(part 1 of 2)
# Autodesk Inventor assembly: Pauk
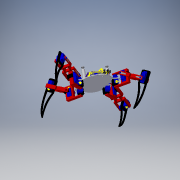
[picture p0: Inventor's stored thumbnail of the model, 180x180]
Saved by Autodesk Inventor 2019 (Build 230136000, 136)
## iProperties
Created: 2018-11-25
Part Number: Pauk
Document SubType Name: Assembly
Designer: nikol
_MechatronicsProject: <Project Version="1.0"><Path>C:\Users\nikol\Desktop\el.emx</Path><Guid>{C559D3A1-3329-4734-BE8F-63649D4C72C8}</Guid><IPJFileName>C:\Users\Public\Documents\Autodesk\Inventor 2019\Default.ipj</IPJFileName><IPJWorkFolder></IPJWorkFolder><AssemblyFileName>C:\Users\nikol\Desktop\ArduinoSpider\Modeli\Pauk.iam</AssemblyFileName><AssemblyFileGUID>{1F7FCD52-C9F9-4255-BD89-D36AF9ACCA5F}</AssemblyFileGUID></Project>
_MTAssemblyInfoProperty: <MechatronicsAssembly Version="1.0" ID="{1F7FCD52-C9F9-4255-BD89-D36AF9ACCA5F}"><MechatronicsComponents><MechatronicsComponent FileName="C:\Users\nikol\Desktop\ArduinoSpider\Modeli\SERVOMOTORARDUINO.ipt"><ReferenceKey Document="C:\Users\nikol\Desktop\ArduinoSpider\Modeli\Pauk.iam" Value="2|1|1|0|4|0|0|0|35|0|0|0|" Context="2|0|0|0|1|0|0|0|" ID="{1F7FCD52-C9F9-4255-BD89-D36AF9ACCA5F}"/><Properties><ComponentTag>(SERVOMOTORARDUINO:14)</ComponentTag><TerminalStripTag></TerminalStripTag><TerminalNumberTag></TerminalNumberTag><Installation></Installation><Location></Location><Category></Category><Manufacture></Manufacture><Catalog></Catalog><AssemblyCode></AssemblyCode><Line1></Line1><Line2></Line2><Line3></Line3><ElectricalType></ElectricalType></Properties><OccurrencePath><Occurrence Name="SERVOMOTORARDUINO:14" FileName="C:\Users\nikol\Desktop\ArduinoSpider\Modeli\SERVOMOTORARDUINO.ipt"/></OccurrencePath></MechatronicsComponent><MechatronicsComponent FileName="C:\Users\nikol\Desktop\ArduinoSpider\Modeli\SERVOMOTORARDUINO.ipt"><ReferenceKey Document="C:\Users\nikol\Desktop\ArduinoSpider\Modeli\Pauk.iam" Value="2|1|1|0|4|0|0|0|34|0|0|0|" Context="2|0|0|0|1|0|0|0|" ID="{1F7FCD52-C9F9-4255-BD89-D36AF9ACCA5F}"/><Properties><ComponentTag>(SERVOMOTORARDUINO:13)</ComponentTag><TerminalStripTag></TerminalStripTag><TerminalNumberTag></TerminalNumberTag><Installation></Installation><Location></Location><Category></Category><Manufacture></Manufacture><Catalog></Catalog><AssemblyCode></AssemblyCode><Line1></Line1><Line2></Line2><Line3></Line3><ElectricalType></ElectricalType></Properties><OccurrencePath><Occurrence Name="SERVOMOTORARDUINO:13" FileName="C:\Users\nikol\Desktop\ArduinoSpider\Modeli\SERVOMOTORARDUINO.ipt"/></OccurrencePath></MechatronicsComponent><MechatronicsComponent FileName="C:\Users\nikol\Desktop\ArduinoSpider\Modeli\SERVOMOTORARDUINO.ipt"><ReferenceKey Document="C:\Users\nikol\Desktop\ArduinoSpider\Modeli\Pauk.iam" Value="2|1|1|0|4|0|0|0|33|0|0|0|" Context="2|0|0|0|1|0|0|0|" ID="{1F7FCD52-C9F9-4255-BD89-D36AF9ACCA5F}"/><Properties><ComponentTag>(SERVOMOTORARDUINO:12)</ComponentTag><TerminalStripTag></TerminalStripTag><TerminalNumberTag></TerminalNumberTag><Installation></Installation><Location></Location><Category></Category><Manufacture></Manufacture><Catalog></Catalog><AssemblyCode></AssemblyCode><Line1></Line1><Line2></Line2><Line3></Line3><ElectricalType></ElectricalType></Properties><OccurrencePath><Occurrence Name="SERVOMOTORARDUINO:12" FileName="C:\Users\nikol\Desktop\ArduinoSpider\Modeli\SERVOMOTORARDUINO.ipt"/></OccurrencePath></MechatronicsComponent><MechatronicsComponent FileName="C:\Users\nikol\Desktop\ArduinoSpider\Modeli\SERVOMOTORARDUINO.ipt"><ReferenceKey Document="C:\Users\nikol\Desktop\ArduinoSpider\Modeli\Pauk.iam" Value="2|1|1|0|4|0|0|0|32|0|0|0|" Context="2|0|0|0|1|0|0|0|" ID="{1F7FCD52-C9F9-4255-BD89-D36AF9ACCA5F}"/><Properties><ComponentTag>(SERVOMOTORARDUINO:11)</ComponentTag><TerminalStripTag></TerminalStripTag><TerminalNumberTag></TerminalNumberTag><Installation></Installation><Location></Location><Category></Category><Manufacture></Manufacture><Catalog></Catalog><AssemblyCode></AssemblyCode><Line1></Line1><Line2></Line2><Line3></Line3><ElectricalType></ElectricalType></Properties><OccurrencePath><Occurrence Name="SERVOMOTORARDUINO:11" FileName="C:\Users\nikol\Desktop\ArduinoSpider\Modeli\SERVOMOTORARDUINO.ipt"/></OccurrencePath></MechatronicsComponent><MechatronicsComponent FileName="C:\Users\nikol\Desktop\ArduinoSpider\Modeli\SERVOMOTORARDUINO.ipt"><ReferenceKey Document="C:\Users\nikol\Desktop\ArduinoSpider\Modeli\Pauk.iam" Value="2|1|1|0|4|0|0|0|31|0|0|0|" Context="2|0|0|0|1|0|0|0|" ID="{1F7FCD52-C9F9-4255-BD89-D36AF9ACCA5F}"/><Properties><ComponentTag>(SERVOMOTORARDUINO:10)</ComponentTag><TerminalStripTag></TerminalStripTag><TerminalNumberTag></TerminalNumberTag><Installation></Installation><Location></Location><Category></Category><Manufacture></Manufacture><Catalog></Catalog><AssemblyCode></AssemblyCode><Line1></Line1><Line2></Line2><Line3></Line3><ElectricalType></ElectricalType></Properties><OccurrencePath><Occurrence Name="SERVOMOTORARDUINO:10" FileName="C:\Users\nikol\Desktop\ArduinoSpider\Modeli\SERVOMOTORARDUINO.ipt"/></OccurrencePath></MechatronicsComponent><MechatronicsComponent FileName="C:\Users\nikol\Desktop\ArduinoSpider\Modeli\SERVOMOTORARDUINO.ipt"><ReferenceKey Document="C:\Users\nikol\Desktop\ArduinoSpider\Modeli\Pauk.iam" Value="2|1|1|0|4|0|0|0|22|0|0|0|" Context="2|0|0|0|1|0|0|0|" ID="{1F7FCD52-C9F9-4255-BD89-D36AF9ACCA5F}"/><Properties><ComponentTag>(SERVOMOTORARDUINO:9)</ComponentTag><TerminalStripTag></TerminalStripTag><TerminalNumberTag></TerminalNumberTag><Installation></Installation><Location></Location><Category></Category><Manufacture></Manufacture><Catalog></Catalog><AssemblyCode></AssemblyCode><Line1></Line1><Line2></Line2><Line3></Line3><ElectricalType></ElectricalType></Properties><OccurrencePath><Occurrence Name="SERVOMOTORARDUINO:9" FileName="C:\Users\nikol\Desktop\ArduinoSpider\Modeli\SERVOMOTORARDUINO.ipt"/></OccurrencePath></MechatronicsComponent><MechatronicsComponent FileName="C:\Users\nikol\Desktop\ArduinoSpider\Modeli\SERVOMOTORARDUINO.ipt"><ReferenceKey Document="C:\Users\nikol\Desktop\ArduinoSpider\Modeli\Pauk.iam" Value="2|1|1|0|4|0|0|0|21|0|0|0|" Context="2|0|0|0|1|0|0|0|" ID="{1F7FCD52-C9F9-4255-BD89-D36AF9ACCA5F}"/><Properties><ComponentTag>(SERVOMOTORARDUINO:8)</ComponentTag><TerminalStripTag></TerminalStripTag><TerminalNumberTag></TerminalNumberTag><Installation></Installation><Location></Location><Category></Category><Manufacture></Manufacture><Catalog></Catalog><AssemblyCode></AssemblyCode><Line1></Line1><Line2></Line2><Line3></Line3><ElectricalType></ElectricalType></Properties><OccurrencePath><Occurrence Name="SERVOMOTORARDUINO:8" FileName="C:\Users\nikol\Desktop\ArduinoSpider\Modeli\SERVOMOTORARDUINO.ipt"/></OccurrencePath></MechatronicsComponent><MechatronicsComponent FileName="C:\Users\nikol\Desktop\ArduinoSpider\Modeli\SERVOMOTORARDUINO.ipt"><ReferenceKey Document="C:\Users\nikol\Desktop\ArduinoSpider\Modeli\Pauk.iam" Value="2|1|1|0|4|0|0|0|20|0|0|0|" Context="2|0|0|0|1|0|0|0|" ID="{1F7FCD52-C9F9-4255-BD89-D36AF9ACCA5F}"/><Properties><ComponentTag>(SERVOMOTORARDUINO:7)</ComponentTag><TerminalStripTag></TerminalStripTag><TerminalNumberTag></TerminalNumberTag><Installation></Installation><Location></Location><Category></Category><Manufacture></Manufacture><Catalog></Catalog><AssemblyCode></AssemblyCode><Line1></Line1><Line2></Line2><Line3></Line3><ElectricalType></ElectricalType></Properties><OccurrencePath><Occurrence Name="SERVOMOTORARDUINO:7" FileName="C:\Users\nikol\Desktop\ArduinoSpider\Modeli\SERVOMOTORARDUINO.ipt"/></OccurrencePath></MechatronicsComponent><MechatronicsComponent FileName="C:\Users\nikol\Desktop\ArduinoSpider\Modeli\SERVOMOTORARDUINO.ipt"><ReferenceKey Document="C:\Users\nikol\Desktop\ArduinoSpider\Modeli\Pauk.iam" Value="2|1|1|0|4|0|0|0|2|0|0|0|" Context="2|0|0|0|1|0|0|0|" ID="{1F7FCD52-C9F9-4255-BD89-D36AF9ACCA5F}"/><Properties><ComponentTag>(SERVOMOTORARDUINO:1)</ComponentTag><TerminalStripTag></TerminalStripTag><TerminalNumberTag></TerminalNumberTag><Installation></Installation><Location></Location><Category></Category><Manufacture></Manufacture><Catalog></Catalog><AssemblyCode></AssemblyCode><Line1></Line1><Line2></Line2><Line3></Line3><ElectricalType></ElectricalType></Properties><OccurrencePath><Occurrence Name="SERVOMOTORARDUINO:1" FileName="C:\Users\nikol\Desktop\ArduinoSpider\Modeli\SERVOMOTORARDUINO.ipt"/></OccurrencePath></MechatronicsComponent><MechatronicsComponent FileName="C:\Users\nikol\Desktop\ArduinoSpider\Modeli\SERVOMOTORARDUINO.ipt"><ReferenceKey Document="C:\Users\nikol\Desktop\ArduinoSpider\Modeli\Pauk.iam" Value="2|1|1|0|4|0|0|0|3|0|0|0|" Context="2|0|0|0|1|0|0|0|" ID="{1F7FCD52-C9F9-4255-BD89-D36AF9ACCA5F}"/><Properties><ComponentTag>(SERVOMOTORARDUINO:2)</ComponentTag><TerminalStripTag></TerminalStripTag><TerminalNumberTag></TerminalNumberTag><Installation></Installation><Location></Location><Category></Category><Manufacture></Manufacture><Catalog></Catalog><AssemblyCode></AssemblyCode><Line1></Line1><Line2></Line2><Line3></Line3><ElectricalType></ElectricalType></Properties><OccurrencePath><Occurrence Name="SERVOMOTORARDUINO:2" FileName="C:\Users\nikol\Desktop\ArduinoSpider\Modeli\SERVOMOTORARDUINO.ipt"/></OccurrencePath></MechatronicsComponent><MechatronicsComponent FileName="C:\Users\nikol\Desktop\ArduinoSpider\Modeli\SERVOMOTORARDUINO.ipt"><ReferenceKey Document="C:\Users\nikol\Desktop\ArduinoSpider\Modeli\Pauk.iam" Value="2|1|1|0|4|0|0|0|4|0|0|0|" Context="2|0|0|0|1|0|0|0|" ID="{1F7FCD52-C9F9-4255-BD89-D36AF9ACCA5F}"/><Properties><ComponentTag>(SERVOMOTORARDUINO:3)</ComponentTag><TerminalStripTag></TerminalStripTag><TerminalNumberTag></TerminalNumberTag><Installation></Installation><Location></Location><Category></Category><Manufacture></Manufacture><Catalog></Catalog><AssemblyCode></AssemblyCode><Line1></Line1><Line2></Line2><Line3></Line3><ElectricalType></ElectricalType></Properties><OccurrencePath><Occurrence Name="SERVOMOTORARDUINO:3" FileName="C:\Users\nikol\Desktop\ArduinoSpider\Modeli\SERVOMOTORARDUINO.ipt"/></OccurrencePath></MechatronicsComponent><MechatronicsComponent FileName="C:\Users\nikol\Desktop\ArduinoSpider\Modeli\SERVOMOTORARDUINO.ipt"><ReferenceKey Document="C:\Users\nikol\Desktop\ArduinoSpider\Modeli\Pauk.iam" Value="2|1|1|0|4|0|0|0|5|0|0|0|" Context="2|0|0|0|1|0|0|0|" ID="{1F7FCD52-C9F9-4255-BD89-D36AF9ACCA5F}"/><Properties><ComponentTag>(SERVOMOTORARDUINO:4)</ComponentTag><TerminalStripTag></TerminalStripTag><TerminalNumberTag></TerminalNumberTag><Installation></Installation><Location></Location><Category></Category><Manufacture></Manufacture><Catalog></Catalog><AssemblyCode></AssemblyCode><Line1></Line1><Line2></Line2><Line3></Line3><ElectricalType></ElectricalType></Properties><OccurrencePath><Occurrence Name="SERVOMOTORARDUINO:4" FileName="C:\Users\nikol\Desktop\ArduinoSpider\Modeli\SERVOMOTORARDUINO.ipt"/></OccurrencePath></MechatronicsComponent><MechatronicsComponent FileName="C:\Users\nikol\Desktop\ArduinoSpider\Modeli\Pertinaks.ipt"><ReferenceKey Document="C:\Users\nikol\Desktop\ArduinoSpider\Modeli\Pauk.iam" Value="2|1|1|0|4|0|0|0|70|0|0|0|" Context="2|0|0|0|1|0|0|0|" ID="{1F7FCD52-C9F9-4255-BD89-D36AF9ACCA5F}"/><Properties><ComponentTag>(Pertinaks:1)</ComponentTag><TerminalStripTag></TerminalStripTag><TerminalNumberTag></TerminalNumberTag><Installation></Installation><Location></Location><Category></Category><Manufacture></Manufacture><Catalog></Catalog><AssemblyCode></AssemblyCode><Line1></Line1><Line2></Line2><Line3></Line3><ElectricalType></ElectricalType></Properties><OccurrencePath><Occurrence Name="Pertinaks:1" FileName="C:\Users\nikol\Desktop\ArduinoSpider\Modeli\Pertinaks.ipt"/></OccurrencePath></MechatronicsComponent><MechatronicsComponent FileName="C:\Users\nikol\Desktop\ArduinoSpider\Modeli\Arduino1.ipt"><ReferenceKey Document="C:\Users\nikol\Desktop\ArduinoSpider\Modeli\Pauk.iam" Value="2|1|1|0|4|0|0|0|71|0|0|0|" Context="2|0|0|0|1|0|0|0|" ID="{1F7FCD52-C9F9-4255-BD89-D36AF9ACCA5F}"/><Properties><ComponentTag>(Arduino1:1)</ComponentTag><TerminalStripTag></TerminalStripTag><TerminalNumberTag></TerminalNumberTag><Installation></Installation><Location></Location><Category></Category><Manufacture></Manufacture><Catalog></Catalog><AssemblyCode></AssemblyCode><Line1></Line1><Line2></Line2><Line3></Line3><ElectricalType></ElectricalType></Properties><OccurrencePath><Occurrence Name="Arduino1:1" FileName="C:\Users\nikol\Desktop\ArduinoSpider\Modeli\Arduino1.ipt"/></OccurrencePath></MechatronicsComponent><MechatronicsComponent FileName="C:\Users\nikol\Desktop\ArduinoSpider\Modeli\konektorservomotora.ipt"><ReferenceKey Document="C:\Users\nikol\Desktop\ArduinoSpider\Modeli\Pauk.iam" Value="2|1|1|0|4|0|0|0|75|0|0|0|" Context="2|0|0|0|1|0|0|0|" ID="{1F7FCD52-C9F9-4255-BD89-D36AF9ACCA5F}"/><Properties><ComponentTag>(konektorservomotora:1)</ComponentTag><TerminalStripTag></TerminalStripTag><TerminalNumberTag></TerminalNumberTag><Installation></Installation><Location></Location><Category></Category><Manufacture></Manufacture><Catalog></Catalog><AssemblyCode></AssemblyCode><Line1></Line1><Line2></Line2><Line3></Line3><ElectricalType></ElectricalType></Properties><OccurrencePath><Occurrence Name="konektorservomotora:1" FileName="C:\Users\nikol\Desktop\ArduinoSpider\Modeli\konektorservomotora.ipt"/></OccurrencePath></MechatronicsComponent><MechatronicsComponent FileName="C:\Users\nikol\Desktop\ArduinoSpider\Modeli\konektorservomotora.ipt"><ReferenceKey Document="C:\Users\nikol\Desktop\ArduinoSpider\Modeli\Pauk.iam" Value="2|1|1|0|4|0|0|0|76|0|0|0|" Context="2|0|0|0|1|0|0|0|" ID="{1F7FCD52-C9F9-4255-BD89-D36AF9ACCA5F}"/><Properties><ComponentTag>(konektorservomotora:2)</ComponentTag><TerminalStripTag></TerminalStripTag><TerminalNumberTag></TerminalNumberTag><Installation></Installation><Location></Location><Category></Category><Manufacture></Manufacture><Catalog></Catalog><AssemblyCode></AssemblyCode><Line1></Line1><Line2></Line2><Line3></Line3><ElectricalType></ElectricalType></Properties><OccurrencePath><Occurrence Name="konektorservomotora:2" FileName="C:\Users\nikol\Desktop\ArduinoSpider\Modeli\konektorservomotora.ipt"/></OccurrencePath></MechatronicsComponent><MechatronicsComponent FileName="C:\Users\nikol\Desktop\ArduinoSpider\Modeli\konektorservomotora.ipt"><ReferenceKey Document="C:\Users\nikol\Desktop\ArduinoSpider\Modeli\Pauk.iam" Value="2|1|1|0|4|0|0|0|78|0|0|0|" Context="2|0|0|0|1|0|0|0|" ID="{1F7FCD52-C9F9-4255-BD89-D36AF9ACCA5F}"/><Properties><ComponentTag>(konektorservomotora:3)</ComponentTag><TerminalStripTag></TerminalStripTag><TerminalNumberTag></TerminalNumberTag><Installation></Installation><Location></Location><Category></Category><Manufacture></Manufacture><Catalog></Catalog><AssemblyCode></AssemblyCode><Line1></Line1><Line2></Line2><Line3></Line3><ElectricalType></ElectricalType></Properties><OccurrencePath><Occurrence Name="konektorservomotora:3" FileName="C:\Users\nikol\Desktop\ArduinoSpider\Modeli\konektorservomotora.ipt"/></OccurrencePath></MechatronicsComponent><MechatronicsComponent FileName="C:\Users\nikol\Desktop\ArduinoSpider\Modeli\konektorservomotora.ipt"><ReferenceKey Document="C:\Users\nikol\Desktop\ArduinoSpider\Modeli\Pauk.iam" Value="2|1|1|0|4|0|0|0|79|0|0|0|" Context="2|0|0|0|1|0|0|0|" ID="{1F7FCD52-C9F9-4255-BD89-D36AF9ACCA5F}"/><Properties><ComponentTag>(konektorservomotora:4)</ComponentTag><TerminalStripTag></TerminalStripTag><TerminalNumberTag></TerminalNumberTag><Installation></Installation><Location></Location><Category></Category><Manufacture></Manufacture><Catalog></Catalog><AssemblyCode></AssemblyCode><Line1></Line1><Line2></Line2><Line3></Line3><ElectricalType></ElectricalType></Properties><OccurrencePath><Occurrence Name="konektorservomotora:4" FileName="C:\Users\nikol\Desktop\ArduinoSpider\Modeli\konektorservomotora.ipt"/></OccurrencePath></MechatronicsComponent><MechatronicsComponent FileName="C:\Users\nikol\Desktop\ArduinoSpider\Modeli\konektorservomotora.ipt"><ReferenceKey Document="C:\Users\nikol\Desktop\ArduinoSpider\Modeli\Pauk.iam" Value="2|1|1|0|4|0|0|0|80|0|0|0|" Context="2|0|0|0|1|0|0|0|" ID="{1F7FCD52-C9F9-4255-BD89-D36AF9ACCA5F}"/><Properties><ComponentTag>(konektorservomotora:5)</ComponentTag><TerminalStripTag></TerminalStripTag><TerminalNumberTag></TerminalNumberTag><Installation></Installation><Location></Location><Category></Category><Manufacture></Manufacture><Catalog></Catalog><AssemblyCode></AssemblyCode><Line1></Line1><Line2></Line2><Line3></Line3><ElectricalType></ElectricalType></Properties><OccurrencePath><Occurrence Name="konektorservomotora:5" FileName="C:\Users\nikol\Desktop\ArduinoSpider\Modeli\konektorservomotora.ipt"/></OccurrencePath></MechatronicsComponent><MechatronicsComponent FileName="C:\Users\nikol\Desktop\ArduinoSpider\Modeli\konektorservomotora.ipt"><ReferenceKey Document="C:\Users\nikol\Desktop\ArduinoSpider\Modeli\Pauk.iam" Value="2|1|1|0|4|0|0|0|81|0|0|0|" Context="2|0|0|0|1|0|0|0|" ID="{1F7FCD52-C9F9-4255-BD89-D36AF9ACCA5F}"/><Properties><ComponentTag>(konektorservomotora:6)</ComponentTag><TerminalStripTag></TerminalStripTag><TerminalNumberTag></TerminalNumberTag><Installation></Installation><Location></Location><Category></Category><Manufacture></Manufacture><Catalog></Catalog><AssemblyCode></AssemblyCode><Line1></Line1><Line2></Line2><Line3></Line3><ElectricalType></ElectricalType></Properties><OccurrencePath><Occurrence Name="konektorservomotora:6" FileName="C:\Users\nikol\Desktop\ArduinoSpider\Modeli\konektorservomotora.ipt"/></OccurrencePath></MechatronicsComponent><MechatronicsComponent FileName="C:\Users\nikol\Desktop\ArduinoSpider\Modeli\konektorservomotora.ipt"><ReferenceKey Document="C:\Users\nikol\Desktop\ArduinoSpider\Modeli\Pauk.iam" Value="2|1|1|0|4|0|0|0|82|0|0|0|" Context="2|0|0|0|1|0|0|0|" ID="{1F7FCD52-C9F9-4255-BD89-D36AF9ACCA5F}"/><Properties><ComponentTag>(konektorservomotora:7)</ComponentTag><TerminalStripTag></TerminalStripTag><TerminalNumberTag></TerminalNumberTag><Installation></Installation><Location></Location><Category></Category><Manufacture></Manufacture><Catalog></Catalog><AssemblyCode></AssemblyCode><Line1></Line1><Line2></Line2><Line3></Line3><ElectricalType></ElectricalType></Properties><OccurrencePath><Occurrence Name="konektorservomotora:7" FileName="C:\Users\nikol\Desktop\ArduinoSpider\Modeli\konektorservomotora.ipt"/></OccurrencePath></MechatronicsComponent><MechatronicsComponent FileName="C:\Users\nikol\Desktop\ArduinoSpider\Modeli\konektorservomotora.ipt"><ReferenceKey Document="C:\Users\nikol\Desktop\ArduinoSpider\Modeli\Pauk.iam" Value="2|1|1|0|4|0|0|0|83|0|0|0|" Context="2|0|0|0|1|0|0|0|" ID="{1F7FCD52-C9F9-4255-BD89-D36AF9ACCA5F}"/><Properties><ComponentTag>(konektorservomotora:8)</ComponentTag><TerminalStripTag></TerminalStripTag><TerminalNumberTag></TerminalNumberTag><Installation></Installation><Location></Location><Category></Category><Manufacture></Manufacture><Catalog></Catalog><AssemblyCode></AssemblyCode><Line1></Line1><Line2></Line2><Line3></Line3><ElectricalType></ElectricalType></Properties><OccurrencePath><Occurrence Name="konektorservomotora:8" FileName="C:\Users\nikol\Desktop\ArduinoSpider\Modeli\konektorservomotora.ipt"/></OccurrencePath></MechatronicsComponent><MechatronicsComponent FileName="C:\Users\nikol\Desktop\ArduinoSpider\Modeli\konektorservomotora.ipt"><ReferenceKey Document="C:\Users\nikol\Desktop\ArduinoSpider\Modeli\Pauk.iam" Value="2|1|1|0|4|0|0|0|84|0|0|0|" Context="2|0|0|0|1|0|0|0|" ID="{1F7FCD52-C9F9-4255-BD89-D36AF9ACCA5F}"/><Properties><ComponentTag>(konektorservomotora:9)</ComponentTag><TerminalStripTag></TerminalStripTag><TerminalNumberTag></TerminalNumberTag><Installation></Installation><Location></Location><Category></Category><Manufacture></Manufacture><Catalog></Catalog><AssemblyCode></AssemblyCode><Line1></Line1><Line2></Line2><Line3></Line3><ElectricalType></ElectricalType></Properties><OccurrencePath><Occurrence Name="konektorservomotora:9" FileName="C:\Users\nikol\Desktop\ArduinoSpider\Modeli\konektorservomotora.ipt"/></OccurrencePath></MechatronicsComponent><MechatronicsComponent FileName="C:\Users\nikol\Desktop\ArduinoSpider\Modeli\konektorservomotora.ipt"><ReferenceKey Document="C:\Users\nikol\Desktop\ArduinoSpider\Modeli\Pauk.iam" Value="2|1|1|0|4|0|0|0|85|0|0|0|" Context="2|0|0|0|1|0|0|0|" ID="{1F7FCD52-C9F9-4255-BD89-D36AF9ACCA5F}"/><Properties><ComponentTag>(konektorservomotora:10)</ComponentTag><TerminalStripTag></TerminalStripTag><TerminalNumberTag></TerminalNumberTag><Installation></Installation><Location></Location><Category></Category><Manufacture></Manufacture><Catalog></Catalog><AssemblyCode></AssemblyCode><Line1></Line1><Line2></Line2><Line3></Line3><ElectricalType></ElectricalType></Properties><OccurrencePath><Occurrence Name="konektorservomotora:10" FileName="C:\Users\nikol\Desktop\ArduinoSpider\Modeli\konektorservomotora.ipt"/></OccurrencePath></MechatronicsComponent><MechatronicsComponent FileName="C:\Users\nikol\Desktop\ArduinoSpider\Modeli\konektorservomotora.ipt"><ReferenceKey Document="C:\Users\nikol\Desktop\ArduinoSpider\Modeli\Pauk.iam" Value="2|1|1|0|4|0|0|0|86|0|0|0|" Context="2|0|0|0|1|0|0|0|" ID="{1F7FCD52-C9F9-4255-BD89-D36AF9ACCA5F}"/><Properties><ComponentTag>(konektorservomotora:11)</ComponentTag><TerminalStripTag></TerminalStripTag><TerminalNumberTag></TerminalNumberTag><Installation></Installation><Location></Location><Category></Category><Manufacture></Manufacture><Catalog></Catalog><AssemblyCode></AssemblyCode><Line1></Line1><Line2></Line2><Line3></Line3><ElectricalType></ElectricalType></Properties><OccurrencePath><Occurrence Name="konektorservomotora:11" FileName="C:\Users\nikol\Desktop\ArduinoSpider\Modeli\konektorservomotora.ipt"/></OccurrencePath></MechatronicsComponent><MechatronicsComponent FileName="C:\Users\nikol\Desktop\ArduinoSpider\Modeli\konektorservomotora.ipt"><ReferenceKey Document="C:\Users\nikol\Desktop\ArduinoSpider\Modeli\Pauk.iam" Value="2|1|1|0|4|0|0|0|87|0|0|0|" Context="2|0|0|0|1|0|0|0|" ID="{1F7FCD52-C9F9-4255-BD89-D36AF9ACCA5F}"/><Properties><ComponentTag>(konektorservomotora:12)</ComponentTag><TerminalStripTag></TerminalStripTag><TerminalNumberTag></TerminalNumberTag><Installation></Installation><Location></Location><Category></Category><Manufacture></Manufacture><Catalog></Catalog><AssemblyCode></AssemblyCode><Line1></Line1><Line2></Line2><Line3></Line3><ElectricalType></ElectricalType></Properties><OccurrencePath><Occurrence Name="konektorservomotora:12" FileName="C:\Users\nikol\Desktop\ArduinoSpider\Modeli\konektorservomotora.ipt"/></OccurrencePath></MechatronicsComponent></MechatronicsComponents><MechatronicsComponentDefs><MechatronicsComponentDef DocInternalName="{2F30AE6A-4756-8F3F-7798-C3836D7B1085}" FileName="C:\Users\nikol\Desktop\ArduinoSpider\Modeli\SERVOMOTORARDUINO.ipt" DocRevID="{DC4BD850-4F92-DFFC-6FAD-EC9EDCE3431F}" iPropertyRevID="{96251C51-68CC-4CA2-A100-1C4D0742D07D}"><Pins><Pin PinIndex="1" PinName="1"/><Pin PinIndex="2" PinName="2"/><Pin PinIndex="3" PinName="3"/></Pins></MechatronicsComponentDef><MechatronicsComponentDef DocInternalName="{0C7EC66A-4FA0-B3DB-CB32-0680520E8217}" FileName="C:\Users\nikol\Desktop\ArduinoSpider\Modeli\Pertinaks.ipt" DocRevID="{95D0E292-4D86-AA93-341C-9680380DBE95}" iPropertyRevID="{173A70C5-9485-4508-83D3-19ED7E3B3132}"><Pins><Pin PinIndex="1" PinName="-"/><Pin PinIndex="2" PinName="+"/></Pins></MechatronicsComponentDef><MechatronicsComponentDef DocInternalName="{33D274B9-454D-7B61-2108-0D977D5D255E}" FileName="C:\Users\nikol\Desktop\ArduinoSpider\Modeli\Arduino1.ipt" DocRevID="{B6A613F3-4FCB-8D10-DDAD-1CB3B4B56157}" iPropertyRevID="{A1C5B445-578A-4FDA-899F-1CD5602A7C9C}"><Pins><Pin PinIndex="1" PinName="0"/><Pin PinIndex="2" PinName="1"/><Pin PinIndex="3" PinName="2"/><Pin PinIndex="4" PinName="3"/><Pin PinIndex="5" PinName="4"/><Pin PinIndex="6" PinName="5"/><Pin PinIndex="7" PinName="6"/><Pin PinIndex="8" PinName="7"/><Pin PinIndex="9" PinName="8"/><Pin PinIndex="10" PinName="9"/><Pin PinIndex="11" PinName="10"/><Pin PinIndex="12" PinName="11"/><Pin PinIndex="13" PinName="12"/><Pin PinIndex="14" PinName="13"/><Pin PinIndex="15" PinName="gnd1"/><Pin PinIndex="16" PinName="aref"/><Pin PinIndex="17" PinName="x"/><Pin PinIndex="18" PinName="y"/><Pin PinIndex="19" PinName="a5"/><Pin PinIndex="20" PinName="a4"/><Pin PinIndex="21" PinName="a3"/><Pin PinIndex="22" PinName="a2"/><Pin PinIndex="23" PinName="a1"/><Pin PinIndex="24" PinName="a0"/><Pin PinIndex="25" PinName="vin"/><Pin PinIndex="26" PinName="gnd2"/><Pin PinIndex="27" PinName="gnd3"/><Pin PinIndex="28" PinName="5v"/><Pin PinIndex="29" PinName="3.3v"/><Pin PinIndex="30" PinName="reset"/><Pin PinIndex="31" PinName="ioref"/><Pin PinIndex="32" PinName="z"/></Pins></MechatronicsComponentDef><MechatronicsComponentDef DocInternalName="{896C2A0A-4C40-C372-D4E0-38A78892474E}" FileName="C:\Users\nikol\Desktop\ArduinoSpider\Modeli\konektorservomotora.ipt" DocRevID="{2BAC76ED-4F6C-BD9C-BFB8-FABEA5BF089B}" iPropertyRevID="{1041DD29-9928-40F7-9F24-75CB1C714556}"><Pins><Pin PinIndex="1" PinName="1"/><Pin PinIndex="2" PinName="2"/><Pin PinIndex="3" PinName="3"/></Pins></MechatronicsComponentDef></MechatronicsComponentDefs><MechatronicsHarnessAssemblies/><MechatronicsConnectionDefs/><MechatronicsConnections/><MechatronicsCableDefs/><MechatronicsCables/><MechatronicsSubAssemblies/><ComponentLinks/><MechatronicsAssemblyRevision FileRevision="42"><Occurrences><Occurrence FileName="C:\Users\nikol\Desktop\ArduinoSpider\Modeli\Arduino1.ipt" Name="Arduino1:1" FileRevision="{4FDFE95B-B5CB-20AF-31BA-53751911C0E3}"/><Occurrence FileName="C:\Users\nikol\Desktop\ArduinoSpider\Modeli\ELISAA.ipt" Name="ELISAA:1" FileRevision="{5EE786FD-C1BC-6D18-A074-A9073208E9E5}"/><Occurrence FileName="C:\Users\nikol\Desktop\ArduinoSpider\Modeli\ELISAA.ipt" Name="ELISAA:10" FileRevision="{5EE786FD-C1BC-6D18-A074-A9073208E9E5}"/><Occurrence FileName="C:\Users\nikol\Desktop\ArduinoSpider\Modeli\ELISAA.ipt" Name="ELISAA:11" FileRevision="{5EE786FD-C1BC-6D18-A074-A9073208E9E5}"/><Occurrence FileName="C:\Users\nikol\Desktop\ArduinoSpider\Modeli\ELISAA.ipt" Name="ELISAA:12" FileRevision="{5EE786FD-C1BC-6D18-A074-A9073208E9E5}"/><Occurrence FileName="C:\Users\nikol\Desktop\ArduinoSpider\Modeli\ELISAA.ipt" Name="ELISAA:2" FileRevision="{5EE786FD-C1BC-6D18-A074-A9073208E9E5}"/><Occurrence FileName="C:\Users\nikol\Desktop\ArduinoSpider\Modeli\ELISAA.ipt" Name="ELISAA:3" FileRevision="{5EE786FD-C1BC-6D18-A074-A9073208E9E5}"/><Occurrence FileName="C:\Users\nikol\Desktop\ArduinoSpider\Modeli\ELISAA.ipt" Name="ELISAA:4" FileRevision="{5EE786FD-C1BC-6D18-A074-A9073208E9E5}"/><Occurrence FileName="C:\Users\nikol\Desktop\ArduinoSpider\Modeli\ELISAA.ipt" Name="ELISAA:5" FileRevision="{5EE786FD-C1BC-6D18-A074-A9073208E9E5}"/><Occurrence FileName="C:\Users\nikol\Desktop\ArduinoSpider\Modeli\ELISAA.ipt" Name="ELISAA:6" FileRevision="{5EE786FD-C1BC-6D18-A074-A9073208E9E5}"/><Occurrence FileName="C:\Users\nikol\Desktop\ArduinoSpider\Modeli\ELISAA.ipt" Name="ELISAA:7" FileRevision="{5EE786FD-C1BC-6D18-A074-A9073208E9E5}"/><Occurrence FileName="C:\Users\nikol\Desktop\ArduinoSpider\Modeli\ELISAA.ipt" Name="ELISAA:8" FileRevision="{5EE786FD-C1BC-6D18-A074-A9073208E9E5}"/><Occurrence FileName="C:\Users\nikol\Desktop\ArduinoSpider\Modeli\ELISAA.ipt" Name="ELISAA:9" FileRevision="{5EE786FD-C1BC-6D18-A074-A9073208E9E5}"/><Occurrence FileName="C:\Users\nikol\Desktop\ArduinoSpider\Modeli\GORE.ipt" Name="GORE:1" FileRevision="{DD720BB1-F762-66D7-2771-AC71970AA562}"/><Occurrence FileName="C:\Users\nikol\Desktop\ArduinoSpider\Modeli\NOGA.ipt" Name="NOGA:1" FileRevision="{72A12C66-7C77-A91E-D7A9-4D1D525B9BC5}"/><Occurrence FileName="C:\Users\nikol\Desktop\ArduinoSpider\Modeli\NOGA.ipt" Name="NOGA:2" FileRevision="{72A12C66-7C77-A91E-D7A9-4D1D525B9BC5}"/><Occurrence FileName="C:\Users\nikol\Desktop\ArduinoSpider\Modeli\NOGA.ipt" Name="NOGA:3" FileRevision="{72A12C66-7C77-A91E-D7A9-4D1D525B9BC5}"/><Occurrence FileName="C:\Users\nikol\Desktop\ArduinoSpider\Modeli\NOGA.ipt" Name="NOGA:4" FileRevision="{72A12C66-7C77-A91E-D7A9-4D1D525B9BC5}"/><Occurrence FileName="C:\Users\nikol\Desktop\ArduinoSpider\Modeli\NOSAC1.ipt" Name="NOSAC1:2" FileRevision="{F5C3C530-D0C0-76CF-BD6C-8884B5D31C4A}"/><Occurrence FileName="C:\Users\nikol\Desktop\ArduinoSpider\Modeli\NOSAC1.ipt" Name="NOSAC1:3" FileRevision="{F5C3C530-D0C0-76CF-BD6C-8884B5D31C4A}"/><Occurrence FileName="C:\Users\nikol\Desktop\ArduinoSpider\Modeli\NOSAC1.ipt" Name="NOSAC1:4" FileRevision="{F5C3C530-D0C0-76CF-BD6C-8884B5D31C4A}"/><Occurrence FileName="C:\Users\nikol\Desktop\ArduinoSpider\Modeli\NOSAC1.ipt" Name="NOSAC1:5" FileRevision="{F5C3C530-D0C0-76CF-BD6C-8884B5D31C4A}"/><Occurrence FileName="C:\Users\nikol\Desktop\ArduinoSpider\Modeli\NOSAC2.ipt" Name="NOSAC2:1" FileRevision="{41E49DF4-637A-BA8B-763F-CD5B0444A474}"/><Occurrence FileName="C:\Users\nikol\Desktop\ArduinoSpider\Modeli\NOSAC2.ipt" Name="NOSAC2:2" FileRevision="{41E49DF4-637A-BA8B-763F-CD5B0444A474}"/><Occurrence FileName="C:\Users\nikol\Desktop\ArduinoSpider\Modeli\NOSAC2.ipt" Name="NOSAC2:3" FileRevision="{41E49DF4-637A-BA8B-763F-CD5B0444A474}"/><Occurrence FileName="C:\Users\nikol\Desktop\ArduinoSpider\Modeli\NOSAC2.ipt" Name="NOSAC2:4" FileRevision="{41E49DF4-637A-BA8B-763F-CD5B0444A474}"/><Occurrence FileName="C:\Users\nikol\Desktop\ArduinoSpider\Modeli\OCI.ipt" Name="OCI:1" FileRevision="{37A46975-7550-7624-D062-34E6DC975DD1}"/><Occurrence FileName="C:\Users\nikol\Desktop\ArduinoSpider\Modeli\OCI.ipt" Name="OCI:2" FileRevision="{37A46975-7550-7624-D062-34E6DC975DD1}"/><Occurrence FileName="C:\Users\nikol\Desktop\ArduinoSpider\Modeli\PODMETAC.ipt" Name="PODMETAC:1" FileRevision="{C659912F-E2BF-4973-A03A-5BC128CA021F}"/><Occurrence FileName="C:\Users\nikol\Desktop\ArduinoSpider\Modeli\PODMETAC.ipt" Name="PODMETAC:2" FileRevision="{C659912F-E2BF-4973-A03A-5BC128CA021F}"/><Occurrence FileName="C:\Users\nikol\Desktop\ArduinoSpider\Modeli\PODMETAC.ipt" Name="PODMETAC:3" FileRevision="{C659912F-E2BF-4973-A03A-5BC128CA021F}"/><Occurrence FileName="C:\Users\nikol\Desktop\ArduinoSpider\Modeli\PODMETAC.ipt" Name="PODMETAC:4" FileRevision="{C659912F-E2BF-4973-A03A-5BC128CA021F}"/><Occurrence FileName="C:\Users\nikol\Desktop\ArduinoSpider\Modeli\PODMETAC2X2.ipt" Name="PODMETAC2X2:1" FileRevision="{4525699C-A40F-3FBA-0928-D4B91D88B7CF}"/><Occurrence FileName="C:\Users\nikol\Desktop\ArduinoSpider\Modeli\PODMETAC2X2.ipt" Name="PODMETAC2X2:2" FileRevision="{4525699C-A40F-3FBA-0928-D4B91D88B7CF}"/><Occurrence FileName="C:\Users\nikol\Desktop\ArduinoSpider\Modeli\PODMETAC2X2.ipt" Name="PODMETAC2X2:3" FileRevision="{4525699C-A40F-3FBA-0928-D4B91D88B7CF}"/><Occurrence FileName="C:\Users\nikol\Desktop\ArduinoSpider\Modeli\PODMETAC2X2.ipt" Name="PODMETAC2X2:4" FileRevision="{4525699C-A40F-3FBA-0928-D4B91D88B7CF}"/><Occurrence FileName="C:\Users\nikol\Desktop\ArduinoSpider\Modeli\PREKIDAC.ipt" Name="PREKIDAC:1" FileRevision="{D67416C0-9D2E-772B-D5F5-6F7DBE31CA98}"/><Occurrence FileName="C:\Users\nikol\Desktop\ArduinoSpider\Modeli\Pertinaks.ipt" Name="Pertinaks:1" FileRevision=""/><Occurrence FileName="C:\Users\nikol\Desktop\ArduinoSpider\Modeli\SERVOMOTORARDUINO.ipt" Name="SERVOMOTORARDUINO:1" FileRevision="{4AC7317C-552E-CAD4-9063-6DCECE89E9E5}"/><Occurrence FileName="C:\Users\nikol\Desktop\ArduinoSpider\Modeli\SERVOMOTORARDUINO.ipt" Name="SERVOMOTORARDUINO:10" FileRevision="{4AC7317C-552E-CAD4-9063-6DCECE89E9E5}"/><Occurrence FileName="C:\Users\nikol\Desktop\ArduinoSpider\Modeli\SERVOMOTORARDUINO.ipt" Name="SERVOMOTORARDUINO:11" FileRevision="{4AC7317C-552E-CAD4-9063-6DCECE89E9E5}"/><Occurrence FileName="C:\Users\nikol\Desktop\ArduinoSpider\Modeli\SERVOMOTORARDUINO.ipt" Name="SERVOMOTORARDUINO:12" FileRevision="{4AC7317C-552E-CAD4-9063-6DCECE89E9E5}"/><Occurrence FileName="C:\Users\nikol\Desktop\ArduinoSpider\Modeli\SERVOMOTORARDUINO.ipt" Name="SERVOMOTORARDUINO:13" FileRevision="{4AC7317C-552E-CAD4-9063-6DCECE89E9E5}"/><Occurrence FileName="C:\Users\nikol\Desktop\ArduinoSpider\Modeli\SERVOMOTORARDUINO.ipt" Name="SERVOMOTORARDUINO:14" FileRevision="{4AC7317C-552E-CAD4-9063-6DCECE89E9E5}"/><Occurrence FileName="C:\Users\nikol\Desktop\ArduinoSpider\Modeli\SERVOMOTORARDUINO.ipt" Name="SERVOMOTORARDUINO:2" FileRevision="{4AC7317C-552E-CAD4-9063-6DCECE89E9E5}"/><Occurrence FileName="C:\Users\nikol\Desktop\ArduinoSpider\Modeli\SERVOMOTORARDUINO.ipt" Name="SERVOMOTORARDUINO:3" FileRevision="{4AC7317C-552E-CAD4-9063-6DCECE89E9E5}"/><Occurrence FileName="C:\Users\nikol\Desktop\ArduinoSpider\Modeli\SERVOMOTORARDUINO.ipt" Name="SERVOMOTORARDUINO:4" FileRevision="{4AC7317C-552E-CAD4-9063-6DCECE89E9E5}"/><Occurrence FileName="C:\Users\nikol\Desktop\ArduinoSpider\Modeli\SERVOMOTORARDUINO.ipt" Name="SERVOMOTORARDUINO:7" FileRevision="{4AC7317C-552E-CAD4-9063-6DCECE89E9E5}"/><Occurrence FileName="C:\Users\nikol\Desktop\ArduinoSpider\Modeli\SERVOMOTORARDUINO.ipt" Name="SERVOMOTORARDUINO:8" FileRevision="{4AC7317C-552E-CAD4-9063-6DCECE89E9E5}"/><Occurrence FileName="C:\Users\nikol\Desktop\ArduinoSpider\Modeli\SERVOMOTORARDUINO.ipt" Name="SERVOMOTORARDUINO:9" FileRevision="{4AC7317C-552E-CAD4-9063-6DCECE89E9E5}"/><Occurrence FileName="C:\Users\nikol\Desktop\ArduinoSpider\Modeli\USTA.ipt" Name="USTA:1" FileRevision="{D5E34D68-7D32-B4EB-8249-C858D6401B2D}"/><Occurrence FileName="C:\Users\nikol\Desktop\ArduinoSpider\Modeli\ZAVRTANJNAJVECI.ipt" Name="ZAVRTANJNAJVECI:1" FileRevision="{E77C00A1-0254-97E6-D6B6-089B311973FA}"/><Occurrence FileName="C:\Users\nikol\Desktop\ArduinoSpider\Modeli\ZAVRTANJNAJVECI.ipt" Name="ZAVRTANJNAJVECI:2" FileRevision="{E77C00A1-0254-97E6-D6B6-089B311973FA}"/><Occurrence FileName="C:\Users\nikol\Desktop\ArduinoSpider\Modeli\ZAVRTANJNAJVECI.ipt" Name="ZAVRTANJNAJVECI:3" FileRevision="{E77C00A1-0254-97E6-D6B6-089B311973FA}"/><Occurrence FileName="C:\Users\nikol\Desktop\ArduinoSpider\Modeli\dolee.ipt" Name="dolee:1" FileRevision="{C7B6E72D-24EB-C810-FFFB-FAF2AB9251E1}"/><Occurrence FileName="C:\Users\nikol\Desktop\ArduinoSpider\Modeli\konektorservomotora.ipt" Name="konektorservomotora:1" FileRevision="{CB19B519-D8E3-0E15-B921-2152EA5511E3}"/><Occurrence FileName="C:\Users\nikol\Desktop\ArduinoSpider\Modeli\konektorservomotora.ipt" Name="konektorservomotora:10" FileRevision="{CB19B519-D8E3-0E15-B921-2152EA5511E3}"/><Occurrence FileName="C:\Users\nikol\Desktop\ArduinoSpider\Modeli\konektorservomotora.ipt" Name="konektorservomotora:11" FileRevision="{CB19B519-D8E3-0E15-B921-2152EA5511E3}"/><Occurrence FileName="C:\Users\nikol\Desktop\ArduinoSpider\Modeli\konektorservomotora.ipt" Name="konektorservomotora:12" FileRevision="{CB19B519-D8E3-0E15-B921-2152EA5511E3}"/><Occurrence FileName="C:\Users\nikol\Desktop\ArduinoSpider\Modeli\konektorservomotora.ipt" Name="konektorservomotora:2" FileRevision="{CB19B519-D8E3-0E15-B921-2152EA5511E3}"/><Occurrence FileName="C:\Users\nikol\Desktop\ArduinoSpider\Modeli\konektorservomotora.ipt" Name="konektorservomotora:3" FileRevision="{CB19B519-D8E3-0E15-B921-2152EA5511E3}"/><Occurrence FileName="C:\Users\nikol\Desktop\ArduinoSpider\Modeli\konektorservomotora.ipt" Name="konektorservomotora:4" FileRevision="{CB19B519-D8E3-0E15-B921-2152EA5511E3}"/><Occurrence FileName="C:\Users\nikol\Desktop\ArduinoSpider\Modeli\konektorservomotora.ipt" Name="konektorservomotora:5" FileRevision="{CB19B519-D8E3-0E15-B921-2152EA5511E3}"/><Occurrence FileName="C:\Users\nikol\Desktop\ArduinoSpider\Modeli\konektorservomotora.ipt" Name="konektorservomotora:6" FileRevision="{CB19B519-D8E3-0E15-B921-2152EA5511E3}"/><Occurrence FileName="C:\Users\nikol\Desktop\ArduinoSpider\Modeli\konektorservomotora.ipt" Name="konektorservomotora:7" FileRevision="{CB19B519-D8E3-0E15-B921-2152EA5511E3}"/><Occurrence FileName="C:\Users\nikol\Desktop\ArduinoSpider\Modeli\konektorservomotora.ipt" Name="konektorservomotora:8" FileRevision="{CB19B519-D8E3-0E15-B921-2152EA5511E3}"/><Occurrence FileName="C:\Users\nikol\Desktop\ArduinoSpider\Modeli\konektorservomotora.ipt" Name="konektorservomotora:9" FileRevision="{CB19B519-D8E3-0E15-B921-2152EA5511E3}"/></Occurrences></MechatronicsAssemblyRevision></MechatronicsAssembly>
Author: nikol
## Documents named in this file (17)
- C:\Users\nikol\Desktop\ArduinoSpider\Modeli\Pauk.iam
- C:\Users\nikol\Desktop\ArduinoSpider\Modeli\dolee.ipt
- C:\Users\nikol\Desktop\ArduinoSpider\Modeli\SERVOMOTORARDUINO.ipt
- C:\Users\nikol\Desktop\ArduinoSpider\Modeli\NOSAC1.ipt
- C:\Users\nikol\Desktop\ArduinoSpider\Modeli\PODMETAC.ipt
- C:\Users\nikol\Desktop\ArduinoSpider\Modeli\PODMETAC2X2.ipt
- C:\Users\nikol\Desktop\ArduinoSpider\Modeli\NOSAC2.ipt
- C:\Users\nikol\Desktop\ArduinoSpider\Modeli\NOGA.ipt
- C:\Users\nikol\Desktop\ArduinoSpider\Modeli\GORE.ipt
- C:\Users\nikol\Desktop\ArduinoSpider\Modeli\USTA.ipt
- C:\Users\nikol\Desktop\ArduinoSpider\Modeli\PREKIDAC.ipt
- C:\Users\nikol\Desktop\ArduinoSpider\Modeli\OCI.ipt
- C:\Users\nikol\Desktop\ArduinoSpider\Modeli\ELISAA.ipt
- C:\Users\nikol\Desktop\ArduinoSpider\Modeli\ZAVRTANJNAJVECI.ipt
- C:\Users\nikol\Desktop\ArduinoSpider\Modeli\Pertinaks.ipt
- C:\Users\nikol\Desktop\ArduinoSpider\Modeli\Arduino1.ipt
- C:\Users\nikol\Desktop\ArduinoSpider\Modeli\konektorservomotora.ipt
## Components (67 placed, 16 different names)
1. dolee:1 — Mate:1, Mate:2, Mate:3, Mate:4, Mate:5, Mate:6, Mate:7, Mate:8, Mate:9, Mate:10, Mate:11, Mate:12, Mate:16, Mate:18, Mate:20, Mate:21, Mate:23, Mate:25, Mate:26, Mate:89, Tangent:5, Tangent:6, Tangent:16, Tangent:17, Tangent:18, Tangent:20, Mate:131, Tangent:21
2. GORE:1 — Mate:89, Angle:14, Mate:90, Mate:92, Mate:93, Tangent:5, Tangent:6, Mate:94, Mate:96, Mate:128, Mate:129, Mate:130
3. ZAVRTANJNAJVECI:1 — Tangent:16, Mate:129
4. ZAVRTANJNAJVECI:2 — Tangent:18, Mate:128
5. ZAVRTANJNAJVECI:3 — Tangent:17, Mate:130
6. SERVOMOTORARDUINO:14 — Mate:75, Tangent:3, Angle:13, Mate:86, Mate:87, Mate:88
7. SERVOMOTORARDUINO:13 — Mate:76, Tangent:4, Angle:12, Mate:83, Mate:84, Mate:85
8. SERVOMOTORARDUINO:12 — Mate:74, Tangent:2, Angle:11, Mate:77, Mate:78, Mate:79
9. SERVOMOTORARDUINO:11 — Mate:73, Tangent:1, Angle:10, Mate:80, Mate:81, Mate:82
10. SERVOMOTORARDUINO:10 — Mate:61, Mate:62, Mate:63, Mate:64, Mate:66, Angle:6
11. SERVOMOTORARDUINO:9 — Mate:36, Mate:37, Mate:38, Mate:39, Mate:52, Mate:72, Angle:9
12. SERVOMOTORARDUINO:8 — Mate:40, Mate:41, Mate:42, Mate:49, Mate:70, Angle:8
13. SERVOMOTORARDUINO:7 — Mate:43, Mate:44, Mate:45, Mate:56, Angle:7
14. SERVOMOTORARDUINO:1 — Mate:10, Mate:11, Mate:12, Mate:14, Mate:15, Mate:35, Angle:5, Angle:14, Mate:95
15. SERVOMOTORARDUINO:2 — Mate:4, Mate:5, Mate:6, Mate:24, Mate:33, Angle:4
16. SERVOMOTORARDUINO:3 — Mate:7, Mate:8, Mate:9, Mate:19, Mate:29, Angle:2
17. SERVOMOTORARDUINO:4 — Mate:1, Mate:2, Mate:3, Mate:22, Mate:31, Angle:3
18. NOSAC1:2 — Mate:27, Mate:29, Angle:2, Mate:36, Mate:37, Mate:38, Mate:39, Mate:53, Mate:54, Mate:109, Tangent:8, Mate:110
19. NOSAC1:3 — Mate:32, Mate:33, Angle:4, Mate:43, Mate:44, Mate:45, Mate:57, Mate:59, Mate:115, Mate:116, Mate:117
20. NOSAC1:4 — Mate:30, Mate:31, Angle:3, Mate:40, Mate:41, Mate:42, Mate:50, Mate:51, Mate:122, Tangent:13, Mate:123
21. NOSAC1:5 — Mate:34, Mate:35, Angle:5, Mate:58, Mate:60, Mate:61, Mate:62, Mate:63, Mate:104, Tangent:7, Mate:105
22. PODMETAC:1 — Mate:14, Mate:15, Mate:16, Mate:34
23. PODMETAC:2 — Mate:18, Mate:19, Mate:20, Mate:27
24. PODMETAC:3 — Mate:24, Mate:25, Mate:26, Mate:32
25. PODMETAC:4 — Mate:21, Mate:22, Mate:23, Mate:30
26. PODMETAC2X2:1 — Mate:52, Mate:53, Mate:54, Mate:71
27. PODMETAC2X2:2 — Mate:49, Mate:50, Mate:51, Mate:69
28. PODMETAC2X2:3 — Mate:56, Mate:57, Mate:59, Mate:67, Mate:68
29. PODMETAC2X2:4 — Mate:58, Mate:60, Mate:64, Mate:65
30. NOSAC2:1 — Mate:67, Mate:68, Angle:7, Mate:75, Tangent:3, Angle:13, Mate:118, Tangent:11, Mate:119, Mate:120, Tangent:12, Mate:121
31. NOSAC2:2 — Mate:65, Mate:66, Angle:6, Mate:76, Tangent:4, Angle:12, Mate:101, Mate:102, Mate:103, Mate:106, Mate:107, Mate:108
32. NOSAC2:3 — Mate:71, Mate:72, Angle:9, Mate:74, Tangent:2, Angle:11, Mate:111, Tangent:9, Mate:112, Mate:113, Tangent:10, Mate:114
33. NOSAC2:4 — Mate:69, Mate:70, Angle:8, Mate:73, Tangent:1, Angle:10, Mate:124, Tangent:14, Mate:125, Mate:126, Tangent:15, Mate:127
34. NOGA:1 — Mate:83, Mate:84, Mate:85
35. NOGA:2 — Mate:86, Mate:87, Mate:88
36. NOGA:3 — Mate:80, Mate:81, Mate:82
37. NOGA:4 — Mate:77, Mate:78, Mate:79
38. USTA:1 — Mate:90, Mate:94, Mate:95, Mate:96, Mate:97, Flush:2
39. PREKIDAC:1 — Mate:92, Mate:93, Mate:97, Mate:98, Mate:99, Flush:1, Mate:100, Flush:3
40. OCI:1 — Mate:98, Mate:99, Flush:1
41. OCI:2 — Mate:100, Flush:2, Flush:3
42. ELISAA:1 — Mate:111, Tangent:9, Mate:112
43. ELISAA:2 — Mate:101, Mate:102, Mate:103
44. ELISAA:3 — Mate:104, Tangent:7, Mate:105
45. ELISAA:4 — Mate:106, Mate:107, Mate:108
46. ELISAA:5 — Mate:113, Tangent:10, Mate:114
47. ELISAA:6 — Mate:115, Mate:116, Mate:117
48. ELISAA:7 — Mate:109, Tangent:8, Mate:110
49. ELISAA:8 — Mate:126, Tangent:15, Mate:127
50. ELISAA:9 — Mate:118, Tangent:11, Mate:119
51. ELISAA:10 — Mate:120, Tangent:12, Mate:121
52. ELISAA:11 — Mate:124, Tangent:14, Mate:125
53. ELISAA:12 — Mate:122, Tangent:13, Mate:123
54. Pertinaks:1 — Mate:132, Flush:4, Flush:5, Mate:133, Mate:134, Mate:135, Flush:6, Flush:7, Flush:8, Mate:136, Mate:137, Flush:11, Mate:138, Flush:13, Mate:139, Flush:15, Mate:140, Flush:17, Mate:141, Mate:142, Flush:19, Flush:21, Mate:143, Flush:23, Mate:144, Mate:145, Flush:25
55. Arduino1:1 — Tangent:20, Mate:131, Tangent:21, Mate:132, Flush:4, Flush:5
56. konektorservomotora:1 — Mate:135, Flush:6, Flush:7, Flush:9
57. konektorservomotora:2 — Flush:8, Mate:136, Flush:9, Flush:10
58. konektorservomotora:3 — Flush:10, Mate:137, Flush:11, Flush:12, Mate:138
59. konektorservomotora:4 — Flush:12, Flush:13, Mate:139, Flush:14
60. konektorservomotora:5 — Flush:14, Flush:15, Mate:140, Flush:16
61. konektorservomotora:6 — Flush:16, Flush:17, Mate:141, Flush:18
62. konektorservomotora:7 — Flush:18, Mate:142, Flush:19, Flush:20
63. konektorservomotora:8 — Flush:20, Flush:21, Mate:143, Flush:22
64. konektorservomotora:9 — Flush:22, Flush:23, Mate:144, Flush:24
65. konektorservomotora:10 — Flush:24, Mate:145, Flush:25, Flush:26, Flush:27, Flush:28
66. konektorservomotora:11 — Flush:26, Flush:27, Flush:28, Flush:29, Flush:30, Flush:31
67. konektorservomotora:12 — Flush:29, Flush:30, Flush:31
## Relationships (201: Mate 137, Flush 31, Tangent 20, Angle 13)
- Mate:1: dolee:1 ↔ SERVOMOTORARDUINO:4
- Mate:2: dolee:1 ↔ SERVOMOTORARDUINO:4
- Mate:3: dolee:1 ↔ SERVOMOTORARDUINO:4
- Mate:4: dolee:1 ↔ SERVOMOTORARDUINO:2
- Mate:5: dolee:1 ↔ SERVOMOTORARDUINO:2
- Mate:6: dolee:1 ↔ SERVOMOTORARDUINO:2
- Mate:7: dolee:1 ↔ SERVOMOTORARDUINO:3
- Mate:8: dolee:1 ↔ SERVOMOTORARDUINO:3
- Mate:9: dolee:1 ↔ SERVOMOTORARDUINO:3
- Mate:10: dolee:1 ↔ SERVOMOTORARDUINO:1
- Mate:11: dolee:1 ↔ SERVOMOTORARDUINO:1
- Mate:12: dolee:1 ↔ SERVOMOTORARDUINO:1
- Mate:14: SERVOMOTORARDUINO:1 ↔ PODMETAC:1
- Mate:15: SERVOMOTORARDUINO:1 ↔ PODMETAC:1
- Mate:16: dolee:1 ↔ PODMETAC:1
- Mate:18: dolee:1 ↔ PODMETAC:2
- Mate:19: SERVOMOTORARDUINO:3 ↔ PODMETAC:2
- Mate:20: dolee:1 ↔ PODMETAC:2
- Mate:21: dolee:1 ↔ PODMETAC:4
- Mate:22: SERVOMOTORARDUINO:4 ↔ PODMETAC:4
- Mate:23: dolee:1 ↔ PODMETAC:4
- Mate:24: SERVOMOTORARDUINO:2 ↔ PODMETAC:3
- Mate:25: dolee:1 ↔ PODMETAC:3
- Mate:26: dolee:1 ↔ PODMETAC:3
- Mate:27: NOSAC1:2 ↔ PODMETAC:2
- Mate:29: SERVOMOTORARDUINO:3 ↔ NOSAC1:2
- Angle:2 (45 deg): SERVOMOTORARDUINO:3 ↔ NOSAC1:2
- Mate:30: NOSAC1:4 ↔ PODMETAC:4
- Mate:31: SERVOMOTORARDUINO:4 ↔ NOSAC1:4
- Angle:3 (225 deg): SERVOMOTORARDUINO:4 ↔ NOSAC1:4
- Mate:32: NOSAC1:3 ↔ PODMETAC:3
- Mate:33: SERVOMOTORARDUINO:2 ↔ NOSAC1:3
- Angle:4 (315 deg): SERVOMOTORARDUINO:2 ↔ NOSAC1:3
- Mate:34: NOSAC1:5 ↔ PODMETAC:1
- Mate:35: SERVOMOTORARDUINO:1 ↔ NOSAC1:5
- Angle:5 (135 deg): SERVOMOTORARDUINO:1 ↔ NOSAC1:5
- Mate:36: SERVOMOTORARDUINO:9 ↔ NOSAC1:2
- Mate:37: SERVOMOTORARDUINO:9 ↔ NOSAC1:2
- Mate:38: SERVOMOTORARDUINO:9 ↔ NOSAC1:2
- Mate:39: SERVOMOTORARDUINO:9 ↔ NOSAC1:2
- Mate:40: SERVOMOTORARDUINO:8 ↔ NOSAC1:4
- Mate:41: SERVOMOTORARDUINO:8 ↔ NOSAC1:4
- Mate:42: SERVOMOTORARDUINO:8 ↔ NOSAC1:4
- Mate:43: SERVOMOTORARDUINO:7 ↔ NOSAC1:3
- Mate:44: SERVOMOTORARDUINO:7 ↔ NOSAC1:3
- Mate:45: SERVOMOTORARDUINO:7 ↔ NOSAC1:3
- Mate:49: SERVOMOTORARDUINO:8 ↔ PODMETAC2X2:2
- Mate:50: NOSAC1:4 ↔ PODMETAC2X2:2
- Mate:51: NOSAC1:4 ↔ PODMETAC2X2:2
- Mate:52: SERVOMOTORARDUINO:9 ↔ PODMETAC2X2:1
- Mate:53: NOSAC1:2 ↔ PODMETAC2X2:1
- Mate:54: NOSAC1:2 ↔ PODMETAC2X2:1
- Mate:56: SERVOMOTORARDUINO:7 ↔ PODMETAC2X2:3
- Mate:57: NOSAC1:3 ↔ PODMETAC2X2:3
- Mate:58: NOSAC1:5 ↔ PODMETAC2X2:4
- Mate:59: NOSAC1:3 ↔ PODMETAC2X2:3
- Mate:60: NOSAC1:5 ↔ PODMETAC2X2:4
- Mate:61: SERVOMOTORARDUINO:10 ↔ NOSAC1:5
- Mate:62: SERVOMOTORARDUINO:10 ↔ NOSAC1:5
- Mate:63: SERVOMOTORARDUINO:10 ↔ NOSAC1:5
- Mate:64: SERVOMOTORARDUINO:10 ↔ PODMETAC2X2:4
- Mate:65: PODMETAC2X2:4 ↔ NOSAC2:2
- Mate:66: SERVOMOTORARDUINO:10 ↔ NOSAC2:2
- Angle:6 (150 deg): SERVOMOTORARDUINO:10 ↔ NOSAC2:2
- Mate:67: PODMETAC2X2:3 ↔ NOSAC2:1
- Mate:68: PODMETAC2X2:3 ↔ NOSAC2:1
- Angle:7 (30 deg): SERVOMOTORARDUINO:7 ↔ NOSAC2:1
- Mate:69: PODMETAC2X2:2 ↔ NOSAC2:4
- Mate:70: SERVOMOTORARDUINO:8 ↔ NOSAC2:4
- Angle:8 (150 deg): SERVOMOTORARDUINO:8 ↔ NOSAC2:4
- Mate:71: PODMETAC2X2:1 ↔ NOSAC2:3
- Mate:72: SERVOMOTORARDUINO:9 ↔ NOSAC2:3
- Angle:9 (30 deg): SERVOMOTORARDUINO:9 ↔ NOSAC2:3
- Mate:73: SERVOMOTORARDUINO:11 ↔ NOSAC2:4
- Tangent:1: SERVOMOTORARDUINO:11 ↔ NOSAC2:4
- Mate:74: SERVOMOTORARDUINO:12 ↔ NOSAC2:3
- Tangent:2: SERVOMOTORARDUINO:12 ↔ NOSAC2:3
- Mate:75: SERVOMOTORARDUINO:14 ↔ NOSAC2:1
- Tangent:3: SERVOMOTORARDUINO:14 ↔ NOSAC2:1
- Mate:76: SERVOMOTORARDUINO:13 ↔ NOSAC2:2
- Tangent:4: SERVOMOTORARDUINO:13 ↔ NOSAC2:2
- Angle:10 (0 deg): SERVOMOTORARDUINO:11 ↔ NOSAC2:4
- Angle:11 (0 deg): SERVOMOTORARDUINO:12 ↔ NOSAC2:3
- Angle:12 (0 deg): SERVOMOTORARDUINO:13 ↔ NOSAC2:2
- Angle:13 (0 deg): SERVOMOTORARDUINO:14 ↔ NOSAC2:1
- Mate:77: SERVOMOTORARDUINO:12 ↔ NOGA:4
- Mate:78: SERVOMOTORARDUINO:12 ↔ NOGA:4
- Mate:79: SERVOMOTORARDUINO:12 ↔ NOGA:4
- Mate:80: SERVOMOTORARDUINO:11 ↔ NOGA:3
- Mate:81: SERVOMOTORARDUINO:11 ↔ NOGA:3
- Mate:82: SERVOMOTORARDUINO:11 ↔ NOGA:3
- Mate:83: SERVOMOTORARDUINO:13 ↔ NOGA:1
- Mate:84: SERVOMOTORARDUINO:13 ↔ NOGA:1
- Mate:85: SERVOMOTORARDUINO:13 ↔ NOGA:1
- Mate:86: SERVOMOTORARDUINO:14 ↔ NOGA:2
- Mate:87: SERVOMOTORARDUINO:14 ↔ NOGA:2
- Mate:88: SERVOMOTORARDUINO:14 ↔ NOGA:2
- Mate:89: dolee:1 ↔ GORE:1
- Angle:14 (0 deg): GORE:1 ↔ SERVOMOTORARDUINO:1
- Mate:90: GORE:1 ↔ USTA:1
- Mate:92: GORE:1 ↔ PREKIDAC:1
- Mate:93: GORE:1 ↔ PREKIDAC:1
- Tangent:5: dolee:1 ↔ GORE:1
- Tangent:6: dolee:1 ↔ GORE:1
- Mate:94: GORE:1 ↔ USTA:1
- Mate:95 (17 mm): SERVOMOTORARDUINO:1 ↔ USTA:1
- Mate:96: GORE:1 ↔ USTA:1
- Mate:97 (3 mm): USTA:1 ↔ PREKIDAC:1
- Mate:98 (5.5 mm): PREKIDAC:1 ↔ OCI:1
- Mate:99 (3 mm): PREKIDAC:1 ↔ OCI:1
- Flush:1: PREKIDAC:1 ↔ OCI:1
- Mate:100 (5.5 mm): PREKIDAC:1 ↔ OCI:2
- Flush:2: USTA:1 ↔ OCI:2
- Flush:3 (-8 mm): PREKIDAC:1 ↔ OCI:2
- Mate:101: NOSAC2:2 ↔ ELISAA:2
- Mate:102: NOSAC2:2 ↔ ELISAA:2
- Mate:103: NOSAC2:2 ↔ ELISAA:2
- Mate:104: NOSAC1:5 ↔ ELISAA:3
- Tangent:7: NOSAC1:5 ↔ ELISAA:3
- Mate:105: NOSAC1:5 ↔ ELISAA:3
- Mate:106: NOSAC2:2 ↔ ELISAA:4
- Mate:107: NOSAC2:2 ↔ ELISAA:4
- Mate:108: NOSAC2:2 ↔ ELISAA:4
- Mate:109: NOSAC1:2 ↔ ELISAA:7
- Tangent:8: NOSAC1:2 ↔ ELISAA:7
- Mate:110: NOSAC1:2 ↔ ELISAA:7
- Mate:111: NOSAC2:3 ↔ ELISAA:1
- Tangent:9: NOSAC2:3 ↔ ELISAA:1
- Mate:112: NOSAC2:3 ↔ ELISAA:1
- Mate:113: NOSAC2:3 ↔ ELISAA:5
- Tangent:10: NOSAC2:3 ↔ ELISAA:5
- Mate:114: NOSAC2:3 ↔ ELISAA:5
- Mate:115: NOSAC1:3 ↔ ELISAA:6
- Mate:116: NOSAC1:3 ↔ ELISAA:6
- Mate:117: NOSAC1:3 ↔ ELISAA:6
- Mate:118: NOSAC2:1 ↔ ELISAA:9
- Tangent:11: NOSAC2:1 ↔ ELISAA:9
- Mate:119: NOSAC2:1 ↔ ELISAA:9
- Mate:120: NOSAC2:1 ↔ ELISAA:10
- Tangent:12: NOSAC2:1 ↔ ELISAA:10
- Mate:121: NOSAC2:1 ↔ ELISAA:10
- Mate:122: NOSAC1:4 ↔ ELISAA:12
- Tangent:13: NOSAC1:4 ↔ ELISAA:12
- Mate:123: NOSAC1:4 ↔ ELISAA:12
- Mate:124: NOSAC2:4 ↔ ELISAA:11
- Tangent:14: NOSAC2:4 ↔ ELISAA:11
- Mate:125: NOSAC2:4 ↔ ELISAA:11
- Mate:126: NOSAC2:4 ↔ ELISAA:8
- Tangent:15: NOSAC2:4 ↔ ELISAA:8
- Mate:127: NOSAC2:4 ↔ ELISAA:8
- Tangent:16: dolee:1 ↔ ZAVRTANJNAJVECI:1
- Tangent:17: dolee:1 ↔ ZAVRTANJNAJVECI:3
- Tangent:18: dolee:1 ↔ ZAVRTANJNAJVECI:2
- Mate:128: GORE:1 ↔ ZAVRTANJNAJVECI:2
- Mate:129: GORE:1 ↔ ZAVRTANJNAJVECI:1
- Mate:130: GORE:1 ↔ ZAVRTANJNAJVECI:3
- Tangent:20: dolee:1 ↔ Arduino1:1
- Mate:131: dolee:1 ↔ Arduino1:1
- Tangent:21: dolee:1 ↔ Arduino1:1
- Mate:132: Pertinaks:1 ↔ Arduino1:1
- Flush:4 (-0.94 mm): Pertinaks:1 ↔ Arduino1:1
- Flush:5 (-4 mm): Pertinaks:1 ↔ Arduino1:1
- Mate:133: Pertinaks:1
- Mate:134: Pertinaks:1
- Mate:135: Pertinaks:1 ↔ konektorservomotora:1
- Flush:6 (5 mm): Pertinaks:1 ↔ konektorservomotora:1
- Flush:7 (19 mm): Pertinaks:1 ↔ konektorservomotora:1
- Flush:8 (7.5 mm): Pertinaks:1 ↔ konektorservomotora:2
- Mate:136: Pertinaks:1 ↔ konektorservomotora:2
- Flush:9: konektorservomotora:1 ↔ konektorservomotora:2
- Flush:10: konektorservomotora:2 ↔ konektorservomotora:3
- Mate:137: Pertinaks:1 ↔ konektorservomotora:3
- Flush:11 (10 mm): Pertinaks:1 ↔ konektorservomotora:3
- Flush:12: konektorservomotora:3 ↔ konektorservomotora:4
- Mate:138: Pertinaks:1 ↔ konektorservomotora:3
- Flush:13 (12.5 mm): Pertinaks:1 ↔ konektorservomotora:4
- Mate:139: Pertinaks:1 ↔ konektorservomotora:4
- Flush:14: konektorservomotora:4 ↔ konektorservomotora:5
- Flush:15 (15 mm): Pertinaks:1 ↔ konektorservomotora:5
- Mate:140: Pertinaks:1 ↔ konektorservomotora:5
- Flush:16: konektorservomotora:5 ↔ konektorservomotora:6
- Flush:17 (-17.78 mm): Pertinaks:1 ↔ konektorservomotora:6
- Mate:141: Pertinaks:1 ↔ konektorservomotora:6
- Flush:18: konektorservomotora:6 ↔ konektorservomotora:7
- Mate:142: Pertinaks:1 ↔ konektorservomotora:7
- Flush:19 (20.32 mm): Pertinaks:1 ↔ konektorservomotora:7
- Flush:20: konektorservomotora:7 ↔ konektorservomotora:8